# Autodesk Inventor assembly: arduinobox
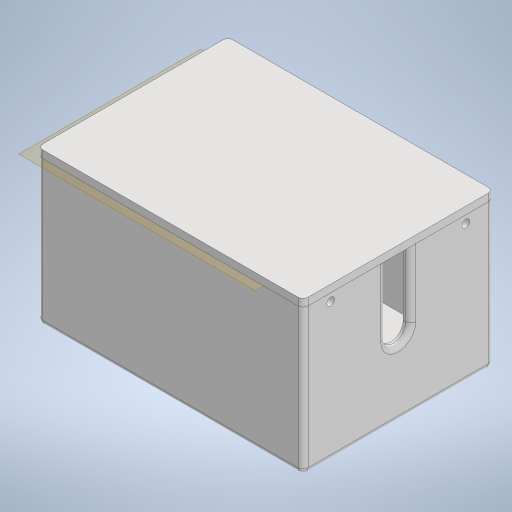
[picture p0: Inventor's stored thumbnail of the model, 512x512]
Saved by Autodesk Inventor 2024 (Build 280153000, 153)
## iProperties
Created: 2024-02-04
Part Number: arduinobox
Document SubType Name: Assembly
Designer: Pavel Povolni
Author: Pavel Povolni
## Documents named in this file (3)
- C:\Users\Pavel Povolni\Desktop\Arbeit\MPI_Promotion\Projektarbeiten\Low Budget Roboter\CAD\Box_Robot_Arduino\Box_Driver.iam
- C:\Users\Pavel Povolni\Desktop\Arbeit\MPI_Promotion\Projektarbeiten\Low Budget Roboter\CAD\Box_Robot_Arduino\Box_Driver_Bottom.ipt
- C:\Users\Pavel Povolni\Desktop\Arbeit\MPI_Promotion\Projektarbeiten\Low Budget Roboter\CAD\Box_Robot_Arduino\Box_Driver_Top.ipt
## Components (2 placed, 2 different names)
1. Box_Driver_Bottom:1 — Fluchtend:1, Fluchtend:2
2. Box_Driver_Top:1 — Fluchtend:1, Fluchtend:2
## Relationships (2: Flush 2)
- Fluchtend:1 [Flush]: Box_Driver_Bottom:1 ↔ Box_Driver_Top:1
- Fluchtend:2 [Flush]: Box_Driver_Bottom:1 ↔ Box_Driver_Top:1
